# Autodesk Inventor assembly: mecanum wheel
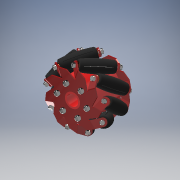
[picture p0: Inventor's stored thumbnail of the model, 180x180]
Saved by Autodesk Inventor 2018 (Build 220112000, 112)
## iProperties
Created: 2023-12-05
Part Number: mecanum wheel
Document SubType Name: Assembly
Designer: DDUGKY
Author: DDUGKY
## Documents named in this file (8)
- C:\Users\DDUGKY\Documents\delwin files\inventor\mecanum wheel\mecanum wheel.iam
- C:\Users\DDUGKY\Documents\delwin files\inventor\mecanum wheel\shaft.ipt
- C:\Users\DDUGKY\Documents\delwin files\inventor\mecanum wheel\body.ipt
- C:\Users\DDUGKY\Documents\delwin files\inventor\mecanum wheel\bolt m3.ipt
- C:\Users\DDUGKY\Documents\delwin files\inventor\mecanum wheel\roller.ipt
- C:\Users\DDUGKY\Documents\delwin files\inventor\mecanum wheel\roller bracket.ipt
- C:\Users\DDUGKY\Documents\delwin files\inventor\mecanum wheel\nut m3.ipt
- C:\Users\DDUGKY\Documents\delwin files\inventor\mecanum wheel\bolt m5.ipt
## Components (60 placed, 7 different names)
1. shaft:1 — Mate:1, Mate:2, Mate:3, Mate:4, Mate:8
2. body:1 — Mate:1, Mate:4, Mate:6, Insert:3, Insert:5, Mate:8
3. body:2 — Mate:2, Mate:3, Mate:5, Mate:7, Insert:4
4. bolt m3:1 — Mate:5, Mate:6, Mate:7
5. nut m3:1 — Insert:3
6. bolt m3:2
7. nut m3:2
8. bolt m3:3 — Rotational:1
9. nut m3:3
10. bolt m3:4
11. nut m3:4
12. bolt m3:5
13. nut m3:5
14. bolt m3:6
15. nut m3:6
16. bolt m3:7
17. nut m3:7
18. bolt m3:8
19. nut m3:8
20. bolt m3:9
21. nut m3:9
22. roller:1 — Insert:1, Insert:2, Rotational:1
23. roller bracket:2 — Insert:1
24. roller bracket:1 — Insert:2
25. roller:2
26. roller bracket:3
27. roller bracket:4
28. roller:3
29. roller bracket:5
30. roller bracket:6
31. roller:4
32. roller bracket:7
33. roller bracket:8
34. roller:5
35. roller bracket:9
36. roller bracket:10
37. roller:6
38. roller bracket:11
39. roller bracket:12
40. roller:7
41. roller bracket:13
42. roller bracket:14
43. roller:8
44. roller bracket:15
45. roller bracket:16
46. roller:9
47. roller bracket:17
48. roller bracket:18
49. bolt m5:2 — Insert:4
50. bolt m5:3
51. bolt m5:4
52. bolt m5:5
53. bolt m5:6
54. bolt m5:7
55. bolt m5:1 — Insert:5
56. bolt m5:8
57. bolt m5:9
58. bolt m5:10
59. bolt m5:11
60. bolt m5:12
## Component patterns: (9 elements, first: bolt m3:1 + nut m3:1), (9 elements, first: roller:1 + roller bracket:2 + roller bracket:1), (6 elements, first: bolt m5:2), (6 elements, first: bolt m5:1)
## Relationships (14: Mate 8, Insert 5, RevoluteJoint 1)
- Mate:1: shaft:1 ↔ body:1
- Mate:2: shaft:1 ↔ body:2
- Mate:3: shaft:1 ↔ body:2
- Mate:4: shaft:1 ↔ body:1
- Mate:5: body:2 ↔ bolt m3:1
- Mate:6: body:1 ↔ bolt m3:1
- Mate:7: body:2 ↔ bolt m3:1
- Insert:1: roller:1 ↔ roller bracket:2
- Insert:2: roller:1 ↔ roller bracket:1
- Insert:3: body:1 ↔ nut m3:1
- Rotational:1 [RevoluteJoint] (-1.5 mm): bolt m3:3 ↔ roller:1
- Insert:4: body:2 ↔ bolt m5:2
- Insert:5: body:1 ↔ bolt m5:1
- Mate:8: shaft:1 ↔ body:1
